# Autodesk Inventor assembly: Bedienhebel
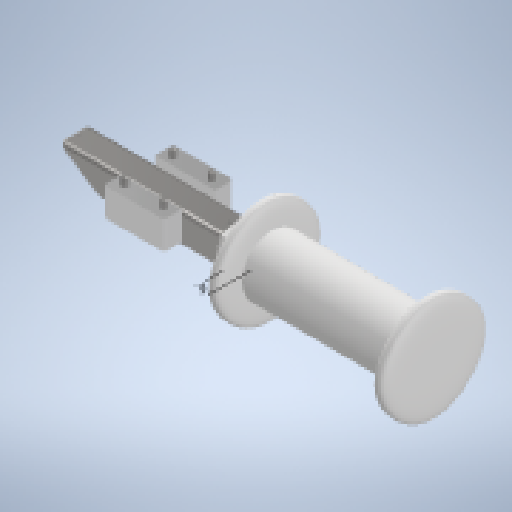
[picture p0: Inventor's stored thumbnail of the model, 512x512]
Saved by Autodesk Inventor 2025 (Build 290162010, 162A)
## iProperties
Created: 2024-11-27
Part Number: Bedienhebel
Document SubType Name: Assembly
Designer: Admin
Author: Admin
## Documents named in this file (10)
- C:\Users\Admin\GIT\HDVKBM\CAD\Krandemonstrator\Bedienhebel.iam
- C:\Users\Admin\GIT\HDVKBM\CAD\Krandemonstrator\HebelhalterBlock.ipt
- C:\Users\Admin\GIT\HDVKBM\CAD\Krandemonstrator\HebelhalterBlockBlind.ipt
- C:\Users\Admin\GIT\HDVKBM\CAD\Krandemonstrator\ISO 12633-2 - 20x20x2 - 200.ipt
- C:\Users\Admin\Documents\Inventor\Content Center Files\R2025\de-DE\DIN 7991(2)\DIN 7991 - M4x40.ipt
- C:\Users\Admin\Documents\Inventor\Content Center Files\R2025\de-DE\AS 1237 (2.1)\AS 1237 - 4.ipt
- C:\Users\Admin\GIT\HDVKBM\CAD\Krandemonstrator\Lagerhülse 6x4x0.ipt
- C:\Users\Admin\Documents\Inventor\Content Center Files\R2025\de-DE\DIN 7991(2)\DIN 7991 - M4x25.ipt
- C:\Users\Admin\GIT\HDVKBM\CAD\Krandemonstrator\knaufErgo.ipt
- C:\Users\Admin\Documents\Inventor\Content Center Files\R2025\de-DE\DIN 7991(2)\DIN 7991 - M3x30.ipt
## Components (13 placed, 9 different names)
1. HebelhalterBlock:1 — Passend:1, Passend:2, Passend:5, Starr:3, Starr:5
2. HebelhalterBlockBlind:1 — Passend:3, Passend:4, Starr:4, Starr:5, Drehbar:1
3. DIN 7991 M4x25:1 — Passend:1
4. DIN 7991 M4x25:2 — Passend:2
5. DIN 7991 M4x25:3 — Passend:3
6. DIN 7991 M4x25:4 — Passend:4
7. DIN 7991 M4x40:1 — Passend:5
8. ISO 12633-2 - 20x20x2 - 200:1 — Drehbar:1, Drehbar:2, Verschiebbar:1, Zylindrisch:1
9. AS 1237 (2.1) 4:1 — Starr:4
10. AS 1237 (2.1) 4:2 — Starr:3
11. Lagerhülse 6x4x0:1 — Drehbar:2
12. knaufErgo:1 — Starr:6, Verschiebbar:1
13. DIN 7991 M3x30:1 — Starr:6, Zylindrisch:1
## Relationships (13: Mate 5, WeldJoint 4, RevoluteJoint 2, TranslationJoint 1, CylindricalJoint 1)
- Passend:1 [Mate]: HebelhalterBlock:1 ↔ DIN 7991 M4x25:1
- Passend:2 [Mate]: HebelhalterBlock:1 ↔ DIN 7991 M4x25:2
- Passend:3 [Mate]: HebelhalterBlockBlind:1 ↔ DIN 7991 M4x25:3
- Passend:4 [Mate]: HebelhalterBlockBlind:1 ↔ DIN 7991 M4x25:4
- Passend:5 [Mate]: HebelhalterBlock:1 ↔ DIN 7991 M4x40:1
- Starr:3 [WeldJoint]: HebelhalterBlock:1 ↔ AS 1237 (2.1) 4:2
- Drehbar:1 [RevoluteJoint] (1 mm): HebelhalterBlockBlind:1 ↔ ISO 12633-2 - 20x20x2 - 200:1
- Starr:4 [WeldJoint]: HebelhalterBlockBlind:1 ↔ AS 1237 (2.1) 4:1
- Starr:5 [WeldJoint] (-22 mm): HebelhalterBlock:1 ↔ HebelhalterBlockBlind:1
- Drehbar:2 [RevoluteJoint]: ISO 12633-2 - 20x20x2 - 200:1 ↔ Lagerhülse 6x4x0:1
- Starr:6 [WeldJoint]: knaufErgo:1 ↔ DIN 7991 M3x30:1
- Verschiebbar:1 [TranslationJoint]: ISO 12633-2 - 20x20x2 - 200:1 ↔ knaufErgo:1
- Zylindrisch:1 [CylindricalJoint]: ISO 12633-2 - 20x20x2 - 200:1 ↔ DIN 7991 M3x30:1
